# Autodesk Inventor assembly: Coins superieur
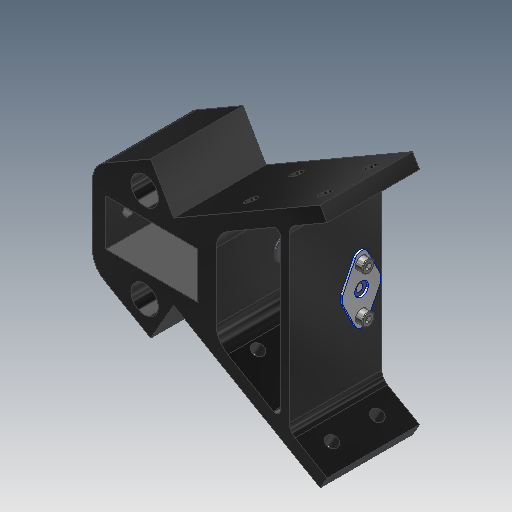
[picture p0: Inventor's stored thumbnail of the model, 512x512]
Saved by Autodesk Inventor 2017 (Build 210142000, 142)
## iProperties
Part Number: Coins superieur
Material: Générique
Document SubType Name: Assembly
Mass: 285.186 g
Surface Area: 396.777 cm^2
Volume: 103.905 cm^3
Density: 2.74469 g/cm^3
Stock Number: 1420-01-15
Project: 1420 Vauban 3D XL
## Documents named in this file (6)
- W:\Professionnel\Conception FABLAB\1420-Vauban 3D XL\1420-01 Armature\1420-01-15 Coins superieur.iam
- W:\Professionnel\Conception FABLAB\1420-Vauban 3D XL\1420-01 Armature\1420-01-04 Coins superieur.ipt
- W:\Professionnel\Conception FABLAB\1420-Vauban 3D XL\1420-01 Armature\1420-01-06 Roulement a bille F623ZZ.ipt
- W:\Professionnel\Conception FABLAB\1420-Vauban 3D XL\1420-01 Armature\1420-01-07 Axe de renvoie.ipt
- W:\Professionnel\Conception FABLAB\1420-Vauban 3D XL\1420-01 Armature\1420-01-08 Maintient roulement.ipt
- W:\Professionnel\Conception FABLAB\1420-Vauban 3D XL\1420-90 Centre de contenu\fr-FR\ANSI B18.3.1M(1)\ANSI B18.3.1M - M3x0,5 x 10(2).ipt
## Components (7 placed, 5 different names)
1. 1420-01-04 Coins superieur:1 — Placage:1, Placage:2, Placage:3, Placage:4, Placage:7, Placage:8, Placage:9, Placage:11, Placage:12
2. 1420-01-06 Roulement a bille F623ZZ:1 — Placage:1, Placage:4, Placage:6
3. 1420-01-06 Roulement a bille F623ZZ:2 — Placage:2, Placage:3, Placage:5
4. 1420-01-07 Axe de renvoie:1 — Placage:5, Placage:6
5. 1420-01-08 Maintient roulement:1 — Placage:7, Placage:8, Placage:9, Placage:10
6. Vis à tête percée - Métrique M3x0,5 x 10:1 — Affleurement:1, Placage:10, Placage:12
7. Vis à tête percée - Métrique M3x0,5 x 10:2 — Affleurement:1, Placage:11
## Relationships (13: Mate 12, Flush 1)
- Placage:1 [Mate]: 1420-01-04 Coins superieur:1 ↔ 1420-01-06 Roulement a bille F623ZZ:1
- Placage:2 [Mate]: 1420-01-04 Coins superieur:1 ↔ 1420-01-06 Roulement a bille F623ZZ:2
- Placage:3 [Mate]: 1420-01-04 Coins superieur:1 ↔ 1420-01-06 Roulement a bille F623ZZ:2
- Placage:4 [Mate]: 1420-01-04 Coins superieur:1 ↔ 1420-01-06 Roulement a bille F623ZZ:1
- Placage:5 [Mate]: 1420-01-06 Roulement a bille F623ZZ:2 ↔ 1420-01-07 Axe de renvoie:1
- Placage:6 [Mate]: 1420-01-06 Roulement a bille F623ZZ:1 ↔ 1420-01-07 Axe de renvoie:1
- Placage:7 [Mate]: 1420-01-04 Coins superieur:1 ↔ 1420-01-08 Maintient roulement:1
- Placage:8 [Mate]: 1420-01-04 Coins superieur:1 ↔ 1420-01-08 Maintient roulement:1
- Placage:9 [Mate]: 1420-01-04 Coins superieur:1 ↔ 1420-01-08 Maintient roulement:1
- Affleurement:1 [Flush]: Vis à tête percée - Métrique M3x0,5 x 10:1 ↔ Vis à tête percée - Métrique M3x0,5 x 10:2
- Placage:10 [Mate]: 1420-01-08 Maintient roulement:1 ↔ Vis à tête percée - Métrique M3x0,5 x 10:1
- Placage:11 [Mate]: 1420-01-04 Coins superieur:1 ↔ Vis à tête percée - Métrique M3x0,5 x 10:2
- Placage:12 [Mate]: 1420-01-04 Coins superieur:1 ↔ Vis à tête percée - Métrique M3x0,5 x 10:1
